# Autodesk Inventor assembly: RuderBauGruppe
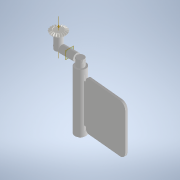
[picture p0: Inventor's stored thumbnail of the model, 180x180]
Saved by Autodesk Inventor 2021 (Build 250183000, 183)
## iProperties
Created: 2021-01-29
Part Number: RuderBauGruppe
Document SubType Name: Assembly
Designer: LETPJG
Author: LETPJG
## Documents named in this file (6)
- C:\Users\LETPJG\Documents\Vault\Gruppen\Gruppe 2\Entwurf\Amphibienfahrzeug\RuderBauGruppe.iam
- C:\Users\LETPJG\Documents\Vault\Gruppen\Gruppe 2\Entwurf\Amphibienfahrzeug\Ruder.ipt
- C:\Users\LETPJG\Documents\Vault\Gruppen\Gruppe 2\Entwurf\Amphibienfahrzeug\KelleWelle3.ipt.iam
- C:\Users\LETPJG\Documents\Vault\Gruppen\Gruppe 2\Entwurf\Amphibienfahrzeug\WellenSchiffsschraube2.ipt
- C:\Users\LETPJG\Documents\Vault\Gruppen\Gruppe 2\Entwurf\Amphibienfahrzeug\BauteilWelle6.ipt
- KelleWelle3.ipt
## Components (4 placed, 4 different names)
1. Ruder:1 — Einfügen:1
2. KelleWelle3.ipt:1 [sub-assembly] — Starr:2
3. WellenSchiffsschraube2:1 — Starr:2, Starr:3
4. BauteilWelle6:1 — Einfügen:1, Starr:3
## Relationships (3: WeldJoint 2, Insert 1)
- Starr:2 [WeldJoint]: KelleWelle3.ipt:1 ↔ WellenSchiffsschraube2:1
- Einfügen:1 [Insert]: Ruder:1 ↔ BauteilWelle6:1
- Starr:3 [WeldJoint]: WellenSchiffsschraube2:1 ↔ BauteilWelle6:1
